# Autodesk Inventor assembly: ASY МОО 001 отстойник осветлитель
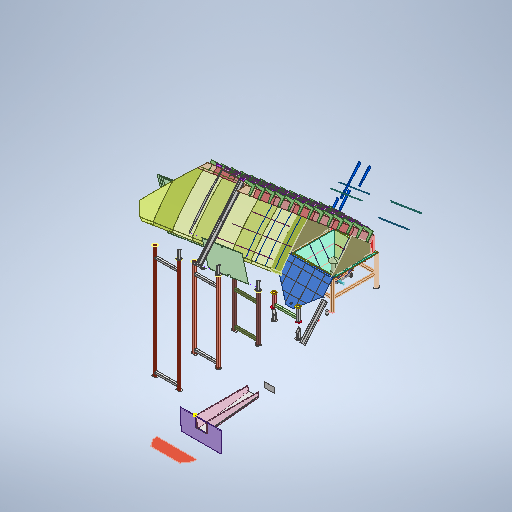
[picture p0: Inventor's stored thumbnail of the model, 512x512]
Saved by Autodesk Inventor 2025 (Build 290162010, 162A)
## iProperties
Created: 2024-04-28
Part Number: ASY МОО 001 отстойник осветлитель
Document SubType Name: Weldment
Designer: admin
Weld Material: Welded Aluminum-6061
Mass: 3.05393e+07 g
Surface Area: 3.06781e+06 cm^2
Volume: 2.84022e+07 cm^3
Density: 1.07525 g/cm^3
Author: admin
## Documents named in this file (68)
- C:\Users\pokla\Documents\Inventor\Отстойник осветлитель\Manturovo_Se-clar-Gleb\ASY MSC 001 отстойник осветлитель.iam
- C:\Users\pokla\Documents\Inventor\Отстойник осветлитель\Manturovo_Se-clar-Gleb\Рама основания\ASY MSC 090 base frame.iam
- C:\Users\pokla\Documents\Inventor\Отстойник осветлитель\Manturovo_Se-clar-Gleb\ASY MSC 010 cone.iam
- C:\Users\pokla\Documents\Inventor\Отстойник осветлитель\Manturovo_Se-clar-Gleb\MSC 000 DIM settler-clarifier.ipt
- C:\Users\pokla\Documents\Inventor\Отстойник осветлитель\Manturovo_Se-clar-Gleb\MSC 031 sheet lowerback.ipt
- C:\Users\pokla\Documents\Inventor\Отстойник осветлитель\Manturovo_Se-clar-Gleb\MSC 021 sheet left board hip.ipt
- C:\Users\pokla\Documents\Inventor\Отстойник осветлитель\Manturovo_Se-clar-Gleb\MSC 022 sheet right board hip.ipt
- C:\Users\pokla\Documents\Inventor\Отстойник осветлитель\Manturovo_Se-clar-Gleb\конус\MSC 071 ridge 1.ipt
- C:\Users\pokla\Documents\Inventor\Отстойник осветлитель\Manturovo_Se-clar-Gleb\конус\MSC 073 ridge 3.ipt
- C:\Users\pokla\Documents\Inventor\Отстойник осветлитель\Manturovo_Se-clar-Gleb\конус\MSC 074 face 1.ipt
- C:\Users\pokla\Documents\Inventor\Отстойник осветлитель\Manturovo_Se-clar-Gleb\Content Center Files\en-US\ISO 5251 B 3D\ISO 5251 Bends 3D without straight ends(90 deg) DN150 11 11.ipt
- C:\Users\pokla\Documents\Inventor\Отстойник осветлитель\Manturovo_Se-clar-Gleb\МОО 061 труба верх 1.ipt
- C:\Users\pokla\Documents\Inventor\Отстойник осветлитель\Manturovo_Se-clar-Gleb\МОО 062 труба верх 2.ipt
- C:\Users\pokla\Documents\Inventor\Отстойник осветлитель\Manturovo_Se-clar-Gleb\МОО 063 труба верх 3.ipt
- C:\Users\pokla\Documents\Inventor\Отстойник осветлитель\Manturovo_Se-clar-Gleb\MSC 0101 sheet gills.ipt
- C:\Users\pokla\Documents\Inventor\Отстойник осветлитель\Manturovo_Se-clar-Gleb\MSC 068 stringer lowerback.ipt
- C:\Users\pokla\Documents\Inventor\Отстойник осветлитель\Manturovo_Se-clar-Gleb\конус\MSC 072 ridge 2.ipt
- C:\Users\pokla\Documents\Inventor\Отстойник осветлитель\Manturovo_Se-clar-Gleb\MSC 075 face 2.ipt
- C:\Users\pokla\Documents\Inventor\Отстойник осветлитель\Manturovo_Se-clar-Gleb\MSC 076 face 3.ipt
- C:\Users\pokla\Documents\Inventor\Отстойник осветлитель\Manturovo_Se-clar-Gleb\MSC 077 face 4.ipt
- C:\Users\pokla\Documents\Inventor\Отстойник осветлитель\Manturovo_Se-clar-Gleb\MSC 035 ring.ipt
- C:\Users\pokla\Documents\Inventor\Отстойник осветлитель\Manturovo_Se-clar-Gleb\MSC 074 ridge 4.ipt
- C:\Users\pokla\Documents\Inventor\Отстойник осветлитель\Manturovo_Se-clar-Gleb\MSC 075 ridge 5.ipt
- C:\Users\pokla\Documents\Inventor\Отстойник осветлитель\Manturovo_Se-clar-Gleb\MSC 081 pillar 1.ipt
- C:\Users\pokla\Documents\Inventor\Отстойник осветлитель\Manturovo_Se-clar-Gleb\MSC 036 flange 500.ipt
- C:\Users\pokla\Documents\Inventor\Отстойник осветлитель\Manturovo_Se-clar-Gleb\MSC 037 flange cover 500.ipt
- C:\Users\pokla\Documents\Inventor\Отстойник осветлитель\Manturovo_Se-clar-Gleb\MSC 038 flange cover ring 500.ipt
- C:\Users\pokla\Documents\Inventor\Отстойник осветлитель\Manturovo_Se-clar-Gleb\MSC 039 flange cover plate 500.ipt
- C:\Users\pokla\Documents\Inventor\Отстойник осветлитель\Manturovo_Se-clar-Gleb\Рама основания\ASY MSC 120  base frame.iam
- C:\Users\pokla\Documents\Inventor\Отстойник осветлитель\Manturovo_Se-clar-Gleb\Рама основания\ASY MSC 121  base frame.iam
- C:\Users\pokla\Documents\Inventor\Отстойник осветлитель\Manturovo_Se-clar-Gleb\Чертеж для парам. рамы.ipt
- C:\Users\pokla\Documents\Inventor\Отстойник осветлитель\Manturovo_Se-clar-Gleb\ASY MSC 120.1  base frame.iam
- C:\Users\pokla\Documents\Inventor\Отстойник осветлитель\Manturovo_Se-clar-Gleb\ASY MSC 122  base frame.iam
- C:\Users\pokla\Documents\Inventor\Отстойник осветлитель\Manturovo_Se-clar-Gleb\ASY MSC 201 BACK.iam
- C:\Users\pokla\Documents\Inventor\Отстойник осветлитель\Manturovo_Se-clar-Gleb\ASY MSC 202 LEFT BOARD.iam
- C:\Users\pokla\Documents\Inventor\Отстойник осветлитель\Manturovo_Se-clar-Gleb\ASY MSC 203 RIGHT BOARD.iam
- C:\Users\pokla\Documents\Inventor\Отстойник осветлитель\Manturovo_Se-clar-Gleb\ASY MSC 204 BELLY.iam
- C:\Users\pokla\Documents\Inventor\Отстойник осветлитель\Manturovo_Se-clar-Gleb\MSC 063 stringer board #.ipt
- C:\Users\pokla\Documents\Inventor\Отстойник осветлитель\Manturovo_Se-clar-Gleb\MSC 064 stringer board ##.ipt
- C:\Users\pokla\Documents\Inventor\Отстойник осветлитель\Manturovo_Se-clar-Gleb\MSC 055 rib hip 2.ipt
- C:\Users\pokla\Documents\Inventor\Отстойник осветлитель\Manturovo_Se-clar-Gleb\MSC 054 rib hip 1.ipt
- C:\Users\pokla\Documents\Inventor\Отстойник осветлитель\Manturovo_Se-clar-Gleb\MSC 0102 sheet gills.ipt
- C:\Users\pokla\Documents\Inventor\Отстойник осветлитель\Manturovo_Se-clar-Gleb\MSC 0202 sheet gills.ipt
- C:\Users\pokla\Documents\Inventor\Отстойник осветлитель\Manturovo_Se-clar-Gleb\MSC 0103 sheet gills.ipt
- C:\Users\pokla\Documents\Inventor\Отстойник осветлитель\Manturovo_Se-clar-Gleb\MSC 0203 sheet gills.ipt
- C:\Users\pokla\Documents\Inventor\Отстойник осветлитель\Manturovo_Se-clar-Gleb\MSC 0104 sheet gills.ipt
- C:\Users\pokla\Documents\Inventor\Отстойник осветлитель\Manturovo_Se-clar-Gleb\MSC 0204 sheet gills.ipt
- C:\Users\pokla\Documents\Inventor\Отстойник осветлитель\Manturovo_Se-clar-Gleb\MSC 0105 sheet gills.ipt
- C:\Users\pokla\Documents\Inventor\Отстойник осветлитель\Manturovo_Se-clar-Gleb\MSC 0205 sheet gills.ipt
- C:\Users\pokla\Documents\Inventor\Отстойник осветлитель\Manturovo_Se-clar-Gleb\MSC 0106 sheet gills.ipt
- C:\Users\pokla\Documents\Inventor\Отстойник осветлитель\Manturovo_Se-clar-Gleb\MSC 0206 sheet gills.ipt
- C:\Users\pokla\Documents\Inventor\Отстойник осветлитель\Manturovo_Se-clar-Gleb\MSC 0107 sheet gills.ipt
- C:\Users\pokla\Documents\Inventor\Отстойник осветлитель\Manturovo_Se-clar-Gleb\MSC 0207 sheet gills.ipt
- C:\Users\pokla\Documents\Inventor\Отстойник осветлитель\Manturovo_Se-clar-Gleb\MSC 079 creen pillar.ipt
- C:\Users\pokla\Documents\Inventor\Отстойник осветлитель\Manturovo_Se-clar-Gleb\ASY MSC 120 support.iam
- C:\Users\pokla\Documents\Inventor\Отстойник осветлитель\Manturovo_Se-clar-Gleb\ракета\МОО 065 ракета труба 5.ipt
- C:\Users\pokla\Documents\Inventor\Отстойник осветлитель\Manturovo_Se-clar-Gleb\ракета\МОО 066 ракета труба 6.ipt
- C:\Users\pokla\Documents\Inventor\Отстойник осветлитель\Manturovo_Se-clar-Gleb\ракета\МОО 067 ракета труба 7.ipt
- C:\Users\pokla\Documents\Inventor\Отстойник осветлитель\Manturovo_Se-clar-Gleb\ракета\МОО 068 ракета труба 8.ipt
- C:\Users\pokla\Documents\Inventor\Отстойник осветлитель\Manturovo_Se-clar-Gleb\MSC 0391 flange.ipt
- C:\Users\pokla\Documents\Inventor\Отстойник осветлитель\Manturovo_Se-clar-Gleb\ASY MSC 0130 cone exit back.iam
- C:\Users\pokla\Documents\Inventor\Отстойник осветлитель\Manturovo_Se-clar-Gleb\MSC DIM 085 tube belly.ipt
- C:\Users\pokla\Documents\Inventor\Отстойник осветлитель\Manturovo_Se-clar-Gleb\MSC 082 pillar 2.ipt
- C:\Users\pokla\Documents\Inventor\Отстойник осветлитель\Manturovo_Se-clar-Gleb\MSC 081 pillar 1_CPY.ipt
- C:\Users\pokla\Documents\Inventor\Отстойник осветлитель\Manturovo_Se-clar-Gleb\MSC 0211 string for sheets.ipt
- C:\Users\pokla\Documents\Inventor\Отстойник осветлитель\Manturovo_Se-clar-Gleb\MSC 0392 flange.ipt
- C:\Users\pokla\Documents\Inventor\Отстойник осветлитель\Manturovo_Se-clar-Gleb\MSC 079 top pillar.ipt
- C:\Users\pokla\Documents\Inventor\BSH_Beshkino_bio_tank\Trommel separator old\MSC DIM 085.1 heel.ipt
## Components (94 placed, 69 different names)
1. MSC 000 DIM settler-clarifier.ipt:1
2. MSC 001 DIM frame.ipt:1 — Flush:94, Mate:95, Mate:97, Mate:99, Mate:100
3. ASY MSC 010 cone.iam:1 [sub-assembly] — Flush:22, Mate:16, Flush:28, Mate:65, Mate:78, Tangent:11, Flush:79, Mate:83, Flush:100, Cylindrical:11
4. ASY MSC 120 support:1 [sub-assembly] — Cylindrical:6
5. ASY MSC 120 support:2 [sub-assembly] — Cylindrical:7
6. ASY MSC 120 support:3 [sub-assembly] — Cylindrical:8
7. ASY MSC 120 support:4 [sub-assembly] — Cylindrical:9
8. ASY MSC 204 BELLY:1 [sub-assembly] — Mate:141, Mate:143, Flush:101, Mate:146, Mate:147, Angle:1
9. ASY MSC 203 RIGHT BOARD:1 [sub-assembly] — Mate:140, Mate:141, Tangent:16, Flush:102
10. ASY MSC 202 LEFT BOARD:1 [sub-assembly] — Mate:142, Mate:143, Tangent:17, Flush:103
11. ASY MSC 201 BACK:1 [sub-assembly] — Mate:134, Tangent:16, Tangent:17
12. ASY MSC 122  base frame:2 [sub-assembly] — Flush:97, Mate:102, Cylindrical:9
13. ASY MSC 120.1  base frame:2 [sub-assembly] — Flush:96, Mate:100, Mate:101, Cylindrical:7
14. ASY MSC 121  base frame:1 [sub-assembly] — Mate:98, Flush:95, Mate:99, Cylindrical:8
15. ASY MSC 120  base frame:1 [sub-assembly] — Flush:93, Mate:97, Cylindrical:6, Cylindrical:10
16. ASY MSC 090 base frame.iam:1 [sub-assembly] — Flush:19, Flush:21, Flush:100
17. MSC 031 sheet lowerback.ipt:1 — Mate:15, Mate:16, Tangent:10, Tangent:11, Tangent:12, Cylindrical:2, Rigid:185, Mate:134
18. MSC 021 sheet left board hip.ipt:1 — Flush:41, Mate:78
19. MSC 022 sheet right board hip.ipt:1 — Mate:30
20. MSC 071 ridge 1.ipt:1 — Mate:50, Rigid:211
21. MSC 073 ridge 3.ipt:1 — Rotational:6, Rigid:210, Rigid:211
22. MSC 072 ridge 2.ipt:1 — Rotational:6
23. MSC 077 face 4.ipt:1
24. MSC 074 ridge 4:1 — Rigid:210
25. MSC 075 ridge 5:1
26. MSC 074 face 1.ipt:1 — Rigid:156, Rigid:157, Flush:62, Rigid:159
27. МОО 061 труба верх 1.ipt:1 — Rigid:59, Rigid:159
28. ISO 5251 Bends 3D without straight ends(90 deg) DN150 11 11.ipt:1 — Rigid:59, Rotational:2
29. МОО 062 труба верх 2.ipt:1 — Rigid:156
30. МОО 063 труба верх 3.ipt:1 — Rigid:157, Rigid:213
31. MSC 068 stringer lowerback.ipt:1 — Mate:65, Tangent:10
32. МОО 061 труба верх 1.ipt:2 — Rotational:2
33. MSC 075 face 2.ipt:1 — Flush:61
34. MSC 076 face 3.ipt:1 — Flush:76
35. MSC 068 stringer lowerback:2 — Mate:83, Tangent:12
36. MSC 035 ring:1 — Cylindrical:2, Rigid:185, Rigid:186
37. MSC 036 flange 500:1 — Rigid:175
38. MSC 036 flange 500:2 — Rigid:175, Rigid:176, Rigid:186
39. MSC 036 flange 500:3 — Rigid:176, Rigid:177, Mate:87
40. MSC 036 flange 500:4 — Rigid:177, Rotational:4
41. MSC 037 flange cover 500:1 — Rotational:4, Mate:87, Rigid:178, Mate:108
42. MSC 038 flange cover ring 500:1 — Rigid:178, Mate:109, Tangent:15
43. MSC 055 rib hip 2:2
44. MSC 063 stringer board #.ipt:2
45. MSC 064 stringer board ##.ipt:2
46. MSC 054 rib board hip 1:2
47. MSC 063 stringer board #.ipt:1
48. MSC 054 rib board hip 1:1
49. MSC 055 rib hip 2:1
50. MSC 064 stringer board ##.ipt:1
51. MSC 0102 sheet gills:1 — Rigid:197, Mate:124, Mate:144, Flush:104, Flush:110
52. MSC 0202 sheet gills:1 — Rigid:197
53. MSC 0103 sheet gills:1 — Rigid:199, Mate:123, Mate:124, Flush:104, Flush:110, Flush:112
54. MSC 0203 sheet gills:1 — Rigid:199
55. MSC 0104 sheet gills:1 — Rigid:201, Mate:122, Mate:123, Flush:107, Flush:112, Flush:113
56. MSC 0204 sheet gills:1 — Rigid:201
57. MSC 0105 sheet gills:1 — Rigid:203, Mate:121, Mate:122, Flush:107, Flush:108, Flush:113, Flush:114
58. MSC 0205 sheet gills:1 — Rigid:203
59. MSC 0106 sheet gills:1 — Rigid:205, Mate:120, Mate:121, Flush:108, Flush:109, Flush:114, Flush:115
60. MSC 0206 sheet gills:1 — Rigid:205
61. MSC 0107 sheet gills:1 — Rigid:206, Mate:120, Flush:109, Flush:115
62. MSC 0207 sheet gills:1 — Rigid:206
63. МОО 065 ракета труба 5:1 — Rigid:209, Rotational:8
64. МОО 066 ракета труба 6:1
65. МОО 067 ракета труба 7:1 — Rigid:209
66. МОО 068 ракета труба 8:1 — Cylindrical:11
67. ASY MSC 120 support:5 [sub-assembly] — Cylindrical:10
68. MSC 0391 flange:1 — Rotational:8
69. ASY MSC 0130 cone exit back:1 [sub-assembly] — Mate:140, Mate:142, Flush:101, Flush:102, Flush:103
70. MSC 0101 sheet gills.ipt:1 — Mate:144
71. MSC 082 pillar 2:1
72. MSC DIM 085 tube belly:1 — Mate:146, Mate:147, Mate:145, Flush:118, Rigid:214, Rigid:215
73. MSC 0101 sheet gills:2 — Tangent:18, Tangent:19, Tangent:20, Angle:1
74. MSC 0392 flange:1 — Rigid:213
75. MSC 079 creen pillar:2 — Mate:148, Rotational:9, Flush:150, Mate:150
76. MSC 081 pillar 1_CPY:1 — Rigid:212, Mate:149, Flush:151
77. MSC 081 pillar 1:1 — Mate:145, Flush:116, Rigid:212, Mate:148, Rotational:10, Flush:118, Flush:150
78. MSC 0211 string for sheets:1 — Rotational:10, Tangent:20
79. MSC 0211 string for sheets:2 — Rotational:9, Tangent:18, Tangent:19
80. MSC 079 top pillar:1 — Mate:149, Flush:151, Mate:150
81. MSC DIM 085.1 heel:1 — Rigid:214
82. MSC DIM 085.1 heel:2 — Rigid:215
83. MSC 039 flange cover plate 500:1 — Mate:108, Mate:109, Tangent:15
84. MSC 039 flange cover plate 500:2
85. MSC 039 flange cover plate 500:3
86. MSC 039 flange cover plate 500:4
87. MSC 039 flange cover plate 500:5
88. MSC 039 flange cover plate 500:6
89. MSC 039 flange cover plate 500:7
90. MSC 039 flange cover plate 500:8
91. MSC 039 flange cover plate 500:9
92. MSC 039 flange cover plate 500:10
93. MSC 039 flange cover plate 500:11
94. MSC 039 flange cover plate 500:12
## Component patterns: (12 elements, first: MSC 039 flange cover plate 500:1)
## Relationships (119: Mate 38, Flush 33, WeldJoint 25, Tangent 9, CylindricalJoint 7, RevoluteJoint 6, Angle 1)
- [Flush]: ASY MSC 201 BACK:1
- Flush:19: ASY MSC 090 base frame.iam:1
- Flush:21: ASY MSC 090 base frame.iam:1
- Flush:22: ASY MSC 010 cone.iam:1
- [Flush]: ASY MSC 010 cone.iam:1
- Mate:15: MSC 031 sheet lowerback.ipt:1
- Mate:16: ASY MSC 010 cone.iam:1 ↔ MSC 031 sheet lowerback.ipt:1
- Flush:28: ASY MSC 010 cone.iam:1
- Flush:41: MSC 021 sheet left board hip.ipt:1
- Mate:30: MSC 022 sheet right board hip.ipt:1
- Mate:50 (200 mm): MSC 071 ridge 1.ipt:1
- Rigid:59 [WeldJoint]: МОО 061 труба верх 1.ipt:1 ↔ ISO 5251 Bends 3D without straight ends(90 deg) DN150 11 11.ipt:1
- Mate:65: ASY MSC 010 cone.iam:1 ↔ MSC 068 stringer lowerback.ipt:1
- [Mate]: ASY MSC 201 BACK:1 ↔ MSC 068 stringer lowerback.ipt:1
- Tangent:10: MSC 031 sheet lowerback.ipt:1 ↔ MSC 068 stringer lowerback.ipt:1
- Rotational:2 [RevoluteJoint]: ISO 5251 Bends 3D without straight ends(90 deg) DN150 11 11.ipt:1 ↔ МОО 061 труба верх 1.ipt:2
- Flush:61: MSC 075 face 2.ipt:1
- Rigid:156 [WeldJoint]: MSC 074 face 1.ipt:1 ↔ МОО 062 труба верх 2.ipt:1
- Rigid:157 [WeldJoint]: MSC 074 face 1.ipt:1 ↔ МОО 063 труба верх 3.ipt:1
- Flush:62: MSC 074 face 1.ipt:1
- Rigid:159 [WeldJoint] (-200 mm): MSC 074 face 1.ipt:1 ↔ МОО 061 труба верх 1.ipt:1
- Flush:76: MSC 076 face 3.ipt:1
- Mate:78: ASY MSC 010 cone.iam:1 ↔ MSC 021 sheet left board hip.ipt:1
- Tangent:11 (22 mm): ASY MSC 010 cone.iam:1 ↔ MSC 031 sheet lowerback.ipt:1
- Flush:79: ASY MSC 010 cone.iam:1
- Mate:83: ASY MSC 010 cone.iam:1 ↔ MSC 068 stringer lowerback:2
- [Mate]: ASY MSC 201 BACK:1 ↔ MSC 068 stringer lowerback:2
- Tangent:12: MSC 031 sheet lowerback.ipt:1 ↔ MSC 068 stringer lowerback:2
- Rigid:175 [WeldJoint]: MSC 036 flange 500:1 ↔ MSC 036 flange 500:2
- Rigid:176 [WeldJoint]: MSC 036 flange 500:2 ↔ MSC 036 flange 500:3
- Rigid:177 [WeldJoint]: MSC 036 flange 500:3 ↔ MSC 036 flange 500:4
- Cylindrical:2: MSC 031 sheet lowerback.ipt:1 ↔ MSC 035 ring:1
- Rotational:4 [RevoluteJoint]: MSC 036 flange 500:4 ↔ MSC 037 flange cover 500:1
- Mate:87: MSC 036 flange 500:3 ↔ MSC 037 flange cover 500:1
- Rigid:178 [WeldJoint]: MSC 037 flange cover 500:1 ↔ MSC 038 flange cover ring 500:1
- Flush:93 (-3 mm): ASY MSC 120  base frame:1
- [Mate]: ASY MSC 120  base frame:1
- Flush:94: MSC 001 DIM frame.ipt:1
- Mate:95: MSC 001 DIM frame.ipt:1
- Mate:97: MSC 001 DIM frame.ipt:1 ↔ ASY MSC 120  base frame:1
- Mate:98: ASY MSC 121  base frame:1
- Flush:95 (-3 mm): ASY MSC 121  base frame:1
- Mate:99: MSC 001 DIM frame.ipt:1 ↔ ASY MSC 121  base frame:1
- Flush:96 (-3 mm): ASY MSC 120.1  base frame:2
- Mate:100: MSC 001 DIM frame.ipt:1 ↔ ASY MSC 120.1  base frame:2
- Mate:101: ASY MSC 120.1  base frame:2
- Flush:97 (-3 mm): ASY MSC 122  base frame:2
- Mate:102: ASY MSC 122  base frame:2
- Rigid:185 [WeldJoint] (20 mm): MSC 031 sheet lowerback.ipt:1 ↔ MSC 035 ring:1
- Mate:108: MSC 037 flange cover 500:1 ↔ MSC 039 flange cover plate 500:1
- Mate:109: MSC 038 flange cover ring 500:1 ↔ MSC 039 flange cover plate 500:1
- Tangent:15: MSC 038 flange cover ring 500:1 ↔ MSC 039 flange cover plate 500:1
- Rigid:186 [WeldJoint]: MSC 035 ring:1 ↔ MSC 036 flange 500:2
- Rigid:197 [WeldJoint]: MSC 0102 sheet gills:1 ↔ MSC 0202 sheet gills:1
- Rigid:199 [WeldJoint]: MSC 0103 sheet gills:1 ↔ MSC 0203 sheet gills:1
- Rigid:201 [WeldJoint]: MSC 0104 sheet gills:1 ↔ MSC 0204 sheet gills:1
- Rigid:203 [WeldJoint]: MSC 0105 sheet gills:1 ↔ MSC 0205 sheet gills:1
- Rigid:205 [WeldJoint]: MSC 0106 sheet gills:1 ↔ MSC 0206 sheet gills:1
- Rigid:206 [WeldJoint]: MSC 0107 sheet gills:1 ↔ MSC 0207 sheet gills:1
- Mate:120 (50 mm): MSC 0106 sheet gills:1 ↔ MSC 0107 sheet gills:1
- Mate:121 (50 mm): MSC 0105 sheet gills:1 ↔ MSC 0106 sheet gills:1
- Mate:122 (50 mm): MSC 0104 sheet gills:1 ↔ MSC 0105 sheet gills:1
- Mate:123 (50 mm): MSC 0103 sheet gills:1 ↔ MSC 0104 sheet gills:1
- Mate:124 (50 mm): MSC 0102 sheet gills:1 ↔ MSC 0103 sheet gills:1
- [Mate]: ASY MSC 204 BELLY:1 ↔ ASY MSC 0130 cone exit back:1
- Flush:100: ASY MSC 010 cone.iam:1 ↔ ASY MSC 090 base frame.iam:1
- Cylindrical:6: ASY MSC 120 support:1 ↔ ASY MSC 120  base frame:1
- Cylindrical:7: ASY MSC 120 support:2 ↔ ASY MSC 120.1  base frame:2
- Cylindrical:8: ASY MSC 120 support:3 ↔ ASY MSC 121  base frame:1
- Cylindrical:9: ASY MSC 120 support:4 ↔ ASY MSC 122  base frame:2
- Mate:134: ASY MSC 201 BACK:1 ↔ MSC 031 sheet lowerback.ipt:1
- [WeldJoint]: ASY MSC 010 cone.iam:1 ↔ ASY MSC 0130 cone exit back:1
- [WeldJoint]: МОО 067 ракета труба 7:1 ↔ ASY MSC 0130 cone exit back:1
- Rigid:209 [WeldJoint]: МОО 065 ракета труба 5:1 ↔ МОО 067 ракета труба 7:1
- Cylindrical:10: ASY MSC 120  base frame:1 ↔ ASY MSC 120 support:5
- Rotational:6 [RevoluteJoint]: MSC 073 ridge 3.ipt:1 ↔ MSC 072 ridge 2.ipt:1
- Rigid:210 [WeldJoint]: MSC 073 ridge 3.ipt:1 ↔ MSC 074 ridge 4:1
- Rigid:211 [WeldJoint]: MSC 071 ridge 1.ipt:1 ↔ MSC 073 ridge 3.ipt:1
- Rotational:8 [RevoluteJoint]: МОО 065 ракета труба 5:1 ↔ MSC 0391 flange:1
- Cylindrical:11: ASY MSC 010 cone.iam:1 ↔ МОО 068 ракета труба 8:1
- Mate:140: ASY MSC 203 RIGHT BOARD:1 ↔ ASY MSC 0130 cone exit back:1
- Mate:141: ASY MSC 204 BELLY:1 ↔ ASY MSC 203 RIGHT BOARD:1
- Tangent:16: ASY MSC 203 RIGHT BOARD:1 ↔ ASY MSC 201 BACK:1
- Mate:142: ASY MSC 202 LEFT BOARD:1 ↔ ASY MSC 0130 cone exit back:1
- Mate:143: ASY MSC 204 BELLY:1 ↔ ASY MSC 202 LEFT BOARD:1
- Tangent:17: ASY MSC 202 LEFT BOARD:1 ↔ ASY MSC 201 BACK:1
- Flush:101: ASY MSC 204 BELLY:1 ↔ ASY MSC 0130 cone exit back:1
- Flush:102: ASY MSC 203 RIGHT BOARD:1 ↔ ASY MSC 0130 cone exit back:1
- Flush:103: ASY MSC 202 LEFT BOARD:1 ↔ ASY MSC 0130 cone exit back:1
- Mate:144 (50 mm): MSC 0102 sheet gills:1 ↔ MSC 0101 sheet gills.ipt:1
- Flush:104: MSC 0102 sheet gills:1 ↔ MSC 0103 sheet gills:1
- Flush:107: MSC 0104 sheet gills:1 ↔ MSC 0105 sheet gills:1
- Flush:108: MSC 0105 sheet gills:1 ↔ MSC 0106 sheet gills:1
- Flush:109: MSC 0106 sheet gills:1 ↔ MSC 0107 sheet gills:1
- Flush:110: MSC 0102 sheet gills:1 ↔ MSC 0103 sheet gills:1
- Flush:112: MSC 0103 sheet gills:1 ↔ MSC 0104 sheet gills:1
- Flush:113: MSC 0104 sheet gills:1 ↔ MSC 0105 sheet gills:1
- Flush:114: MSC 0105 sheet gills:1 ↔ MSC 0106 sheet gills:1
- Flush:115: MSC 0106 sheet gills:1 ↔ MSC 0107 sheet gills:1
- Mate:145: MSC DIM 085 tube belly:1 ↔ MSC 081 pillar 1:1
- Flush:116: MSC 081 pillar 1:1
- Mate:146 (3 mm): ASY MSC 204 BELLY:1 ↔ MSC DIM 085 tube belly:1
- Mate:147 (3 mm): ASY MSC 204 BELLY:1 ↔ MSC DIM 085 tube belly:1
- Rigid:212 [WeldJoint]: MSC 081 pillar 1_CPY:1 ↔ MSC 081 pillar 1:1
- Mate:148 (635 mm): MSC 079 creen pillar:2 ↔ MSC 081 pillar 1:1
- Rotational:9 [RevoluteJoint] (-5 mm): MSC 079 creen pillar:2 ↔ MSC 0211 string for sheets:2
- Rotational:10 [RevoluteJoint] (-5 mm): MSC 081 pillar 1:1 ↔ MSC 0211 string for sheets:1
- Tangent:18: MSC 0101 sheet gills:2 ↔ MSC 0211 string for sheets:2
- Tangent:19: MSC 0101 sheet gills:2 ↔ MSC 0211 string for sheets:2
- Tangent:20: MSC 0101 sheet gills:2 ↔ MSC 0211 string for sheets:1
- Flush:118: MSC DIM 085 tube belly:1 ↔ MSC 081 pillar 1:1
- Flush:150: MSC 079 creen pillar:2 ↔ MSC 081 pillar 1:1
- Angle:1 (0 deg): ASY MSC 204 BELLY:1 ↔ MSC 0101 sheet gills:2
- Rigid:213 [WeldJoint]: МОО 063 труба верх 3.ipt:1 ↔ MSC 0392 flange:1
- Rigid:214 [WeldJoint]: MSC DIM 085 tube belly:1 ↔ MSC DIM 085.1 heel:1
- Rigid:215 [WeldJoint]: MSC DIM 085 tube belly:1 ↔ MSC DIM 085.1 heel:2
- Mate:149: MSC 081 pillar 1_CPY:1 ↔ MSC 079 top pillar:1
- Flush:151: MSC 081 pillar 1_CPY:1 ↔ MSC 079 top pillar:1
- Mate:150: MSC 079 creen pillar:2 ↔ MSC 079 top pillar:1
## Named parameters: Бак_нахлест_фланца = 25 mm, Шаг_опор_по_баку = 2000 mm
